# Autodesk Inventor assembly: BoubleWheelAssy
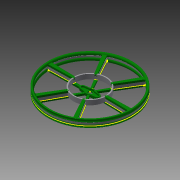
[picture p0: Inventor's stored thumbnail of the model, 180x180]
Saved by Autodesk Inventor 2014 SP1 (Build 180222100, 222)
## iProperties
Created: 2017-01-25
Part Number: BoubleWheelAssy
Document SubType Name: Assembly
Designer: danielsikar
Author: danielsikar
## Documents named in this file (4)
- C:\Users\danielsikar\Documents\Inventor\IoT-Trike\Assemblies\BoubleWheelAssy.iam
- C:\Users\danielsikar\Documents\Inventor\IoT-Trike\Parts\WheelDia190.ipt
- C:\Users\danielsikar\Documents\Inventor\IoT-Trike\Parts\WheelDia190-Top.ipt
- C:\Users\danielsikar\Documents\Inventor\IoT-Trike\Parts\Wheel-190D-Join.ipt
## Components (3 placed, 3 different names)
1. WheelDia190:1 — Mate:1, Mate:2, Mate:3, Mate:4, Flush:1, Flush:3
2. WheelDia190-Top:1 — Mate:4, Mate:5, Mate:6, Flush:2
3. Wheel-190D-Join:1 — Flush:1, Flush:2, Flush:3
## Relationships (9: Mate 6, Flush 3)
- Mate:1: WheelDia190:1
- Mate:2: WheelDia190:1
- Mate:3: WheelDia190:1
- Mate:4 (5 mm): WheelDia190:1 ↔ WheelDia190-Top:1
- Mate:5: WheelDia190-Top:1
- Mate:6: WheelDia190-Top:1
- Flush:1: WheelDia190:1 ↔ Wheel-190D-Join:1
- Flush:2: WheelDia190-Top:1 ↔ Wheel-190D-Join:1
- Flush:3: WheelDia190:1 ↔ Wheel-190D-Join:1
